# Autodesk Inventor assembly: FTC Drivetrain V1
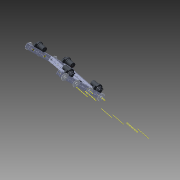
[picture p0: Inventor's stored thumbnail of the model, 180x180]
Saved by Autodesk Inventor 2015 (Build 190159000, 159)
## iProperties
Created: 2014-08-16
Part Number: FTC Drivetrain V1
Document SubType Name: Assembly
Designer: Vinay
Author: Vinay
## Documents named in this file (17)
- C:\Working Folder\FTC Drivetrain V1.iam
- C:\Working Folder\CAD Models\Imported Components\Pitsco Education-739069\Pitsco Education-739069.ipt
- C:\Working Folder\CAD Models\FTC_Tetrix_KOP_Block_Party\Tetrix_Kit_FTC\Imported Components\tetrix_739089_2012\tetrix_739089_2012.ipt
- C:\Working Folder\CAD Models\FTC_Tetrix_KOP_Block_Party\Tetrix_Kit_FTC\Imported Components\tetrix_739083_motor_2012\tetrix_739083_motor_2012.ipt
- C:\Working Folder\CAD Models\Imported Components\Pitsco Education-739091\Pitsco Education-739091.ipt
- C:\Working Folder\CAD Models\Imported Components\Pitsco Education-739069\Pitsco Education-739069_MIR.ipt
- C:\Working Folder\CAD Models\FTC_Tetrix_KOP_Block_Party\Tetrix_Kit_FTC\Imported Components\tetrix_739089_2012\tetrix_739089_2012_MIR.ipt
- C:\Working Folder\CAD Models\FTC_Tetrix_KOP_Block_Party\Tetrix_Kit_FTC\Imported Components\tetrix_739083_motor_2012\tetrix_739083_motor_2012_MIR.ipt
- C:\Working Folder\CAD Models\Imported Components\Pitsco Education-739091\Pitsco Education-739091_MIR.ipt
- C:\Working Folder\CAD Models\FTC_Tetrix_KOP_Block_Party\Tetrix_Kit_FTC\Imported Components\tetrix_739062_2012\tetrix_739062_2012.ipt
- C:\Working Folder\CAD Models\Imported Components\Pitsco Education-739068\Pitsco Education-739068.ipt
- C:\Working Folder\CAD Models\FTC_Tetrix_KOP_Block_Party\Tetrix_Kit_FTC\Imported Components\tetrix_739088_2013\tetrix_739088_2013.ipt
- C:\Working Folder\CAD Models\FTC_Tetrix_KOP_Block_Party\Tetrix_Kit_FTC\Imported Components\tetrix_739079_2012\tetrix_739079_2012.iam
- C:\Working Folder\CAD Models\FTC_Tetrix_KOP_Block_Party\Tetrix_Kit_FTC\Imported Components\tetrix_739172_2012\tetrix_739172_2012.iam
- C:\Working Folder\CAD Models\Imported Components\Pitsco Education-739169\Pitsco Education-739169.ipt
- C:\Working Folder\CAD Models\FTC_Tetrix_KOP_Block_Party\Tetrix_Kit_FTC\Imported Components\tetrix_739165_sprk_25_16t_2013\tetrix_739165_sprk_25_16t_2013.ipt
- C:\Working Folder\CAD Models\FTC_Tetrix_KOP_Block_Party\Tetrix_Kit_FTC\Imported Components\tetrix_739092_2012\tetrix_739092_2012.iam
## Components (72 placed, 16 different names)
1. Pitsco Education-739069:1 — Mate:1, Mate:2, Mate:3, Mate:4, Mate:5, Mate:6, Mate:11, Mate:12, Mate:13, Mate:14, Mate:17, Mate:18, Mate:19, Mate:20, Mate:21, Mate:22, Mate:23, Mate:24, Mate:49, Mate:50, Mate:51, Mate:61, Mate:62, Mate:63, Mate:70, Mate:71, Mate:72, Mate:73
2. tetrix_739089_2012:1 — Mate:4, Mate:5, Mate:6, Mate:7, Flush:2
3. tetrix_739089_2012:2 — Mate:1, Mate:2, Mate:3, Mate:8, Flush:1
4. tetrix_739083_motor_2012:1 — Mate:7, Flush:2, Mate:86, Mate:87
5. tetrix_739083_motor_2012:2 — Mate:8, Flush:1, Mate:88, Mate:89
6. Pitsco Education-739091:1 — Mate:11, Mate:12, Mate:134, Mate:135
7. Pitsco Education-739091:3 — Mate:13, Mate:14, Mate:85, Mate:94
8. Pitsco Education-739091:4 — Mate:72, Mate:73, Mate:82, Mate:100
9. Pitsco Education-739091:5 — Mate:23, Mate:24, Mate:146, Mate:147
10. Pitsco Education-739091:6 — Mate:70, Mate:71, Mate:84, Mate:96
11. Pitsco Education-739091:7 — Mate:21, Mate:22, Mate:142, Mate:143
12. Pitsco Education-739091:10 — Mate:19, Mate:20, Mate:136, Mate:137
13. Pitsco Education-739091:11 — Mate:17, Mate:18, Mate:83, Mate:98
14. Pitsco Education-739069_MIR:1 — Mate:25, Mate:26, Mate:27, Mate:28, Mate:29, Mate:30, Mate:33, Mate:34, Mate:35, Mate:36, Mate:39, Mate:40, Mate:43, Mate:44, Mate:45, Mate:46, Mate:47, Mate:48, Mate:58, Mate:59, Mate:60, Mate:74, Mate:75, Mate:76, Mate:77
15. tetrix_739089_2012_MIR:1 — Mate:25, Mate:26, Mate:27, Flush:3, Mate:31
16. tetrix_739089_2012_MIR:2 — Mate:28, Mate:29, Mate:30, Flush:4, Mate:32
17. tetrix_739083_motor_2012_MIR:1 — Flush:3, Mate:31, Mate:90, Mate:91
18. tetrix_739083_motor_2012_MIR:2 — Flush:4, Mate:32, Mate:92, Mate:93
19. Pitsco Education-739091_MIR:1 — Mate:33, Mate:34, Mate:140, Mate:141
20. Pitsco Education-739091_MIR:2 — Mate:35, Mate:36, Mate:81, Mate:108
21. Pitsco Education-739091_MIR:3 — Mate:76, Mate:77, Mate:78, Mate:106
22. Pitsco Education-739091_MIR:4 — Mate:39, Mate:40, Mate:148, Mate:149
23. Pitsco Education-739091_MIR:5 — Mate:74, Mate:75, Mate:80, Mate:102
24. Pitsco Education-739091_MIR:6 — Mate:43, Mate:44, Mate:144, Mate:145
25. Pitsco Education-739091_MIR:7 — Mate:45, Mate:46, Mate:138, Mate:139
26. Pitsco Education-739091_MIR:8 — Mate:47, Mate:48, Mate:79, Mate:104
27. tetrix_739062_2012:2 — Mate:49, Mate:50, Mate:51, Mate:52, Mate:53, Mate:54
28. Pitsco Education-739068:1 — Mate:52, Mate:53, Mate:54, Mate:55, Mate:56, Mate:57
29. tetrix_739062_2012:5 — Mate:55, Mate:56, Mate:57, Mate:58, Mate:59, Mate:60
30. tetrix_739062_2012:6 — Mate:61, Mate:62, Mate:63, Mate:64, Mate:65, Mate:66
31. tetrix_739062_2012:7 — Mate:67, Mate:68, Mate:69
32. Pitsco Education-739068:2 — Mate:64, Mate:65, Mate:66, Mate:67, Mate:68, Mate:69
33. tetrix_739088_2013:1 — Mate:81, Mate:109, Cylindrical:1
34. tetrix_739088_2013:2 — Mate:80, Mate:103, Mate:150
35. tetrix_739088_2013:3 — Mate:79, Mate:105
36. tetrix_739088_2013:4 — Mate:78, Mate:107
37. tetrix_739088_2013:5 — Mate:85, Mate:95
38. tetrix_739088_2013:6 — Mate:84, Mate:97
39. tetrix_739088_2013:7 — Mate:83, Mate:99
40. tetrix_739088_2013:8 — Mate:82, Mate:101
41. tetrix_739079_2012:1 [sub-assembly] — Mate:88, Mate:89, Mate:112, Mate:113
42. tetrix_739079_2012:2 [sub-assembly] — Mate:86, Mate:87, Mate:116, Mate:117
43. tetrix_739079_2012:3 [sub-assembly] — Mate:92, Mate:93, Mate:122, Mate:123
44. tetrix_739079_2012:4 [sub-assembly] — Mate:90, Mate:91, Mate:132, Mate:133
45. tetrix_739172_2012:1 [sub-assembly] — Mate:94, Mate:95, Mate:110, Mate:111
46. tetrix_739172_2012:2 [sub-assembly] — Mate:100, Mate:101, Mate:120, Mate:121
47. tetrix_739172_2012:3 [sub-assembly] — Mate:98, Mate:99, Mate:118, Mate:119
48. tetrix_739172_2012:4 [sub-assembly] — Mate:96, Mate:97, Mate:114, Mate:115
49. tetrix_739172_2012:5 [sub-assembly] — Mate:102, Mate:103, Mate:128, Mate:129
50. tetrix_739172_2012:6 [sub-assembly] — Mate:104, Mate:105, Mate:126, Mate:127
51. tetrix_739172_2012:7 [sub-assembly] — Mate:106, Mate:107, Mate:124, Mate:125
52. tetrix_739172_2012:8 [sub-assembly] — Mate:108, Mate:109, Mate:130, Mate:131
53. Pitsco Education-739169:1 — Mate:110, Mate:111
54. Pitsco Education-739169:2 — Mate:114, Mate:115
55. Pitsco Education-739169:3 — Mate:118, Mate:119
56. Pitsco Education-739169:4 — Mate:120, Mate:121
57. tetrix_739165_sprk_25_16t_2013:1 — Mate:122, Mate:123
58. tetrix_739165_sprk_25_16t_2013:2 — Mate:112, Mate:113
59. tetrix_739165_sprk_25_16t_2013:3 — Mate:116, Mate:117
60. Pitsco Education-739169:5 — Mate:124, Mate:125
61. Pitsco Education-739169:6 — Mate:126, Mate:127
62. Pitsco Education-739169:7 — Mate:130, Mate:131, Cylindrical:1
63. Pitsco Education-739169:8 — Mate:128, Mate:129
64. tetrix_739165_sprk_25_16t_2013:4 — Mate:132, Mate:133
65. tetrix_739092_2012:1 [sub-assembly] — Mate:138, Mate:139
66. tetrix_739092_2012:2 [sub-assembly] — Mate:142, Mate:143
67. tetrix_739092_2012:3 [sub-assembly] — Mate:140, Mate:141
68. tetrix_739092_2012:4 [sub-assembly] — Mate:146, Mate:147
69. tetrix_739092_2012:5 [sub-assembly] — Mate:136, Mate:137
70. tetrix_739092_2012:6 [sub-assembly] — Mate:144, Mate:145, Mate:150
71. tetrix_739092_2012:7 [sub-assembly] — Mate:148, Mate:149
72. tetrix_739092_2012:8 [sub-assembly] — Mate:134, Mate:135
## Relationships (147: Mate 142, Flush 4, CylindricalJoint 1)
- Mate:1: Pitsco Education-739069:1 ↔ tetrix_739089_2012:2
- Mate:2: Pitsco Education-739069:1 ↔ tetrix_739089_2012:2
- Mate:3: Pitsco Education-739069:1 ↔ tetrix_739089_2012:2
- Mate:4: Pitsco Education-739069:1 ↔ tetrix_739089_2012:1
- Mate:5: Pitsco Education-739069:1 ↔ tetrix_739089_2012:1
- Mate:6: Pitsco Education-739069:1 ↔ tetrix_739089_2012:1
- Mate:7: tetrix_739089_2012:1 ↔ tetrix_739083_motor_2012:1
- Mate:8: tetrix_739089_2012:2 ↔ tetrix_739083_motor_2012:2
- Flush:1: tetrix_739089_2012:2 ↔ tetrix_739083_motor_2012:2
- Flush:2: tetrix_739089_2012:1 ↔ tetrix_739083_motor_2012:1
- Mate:11: Pitsco Education-739069:1 ↔ Pitsco Education-739091:1
- Mate:12: Pitsco Education-739069:1 ↔ Pitsco Education-739091:1
- Mate:13: Pitsco Education-739069:1 ↔ Pitsco Education-739091:3
- Mate:14: Pitsco Education-739069:1 ↔ Pitsco Education-739091:3
- Mate:17: Pitsco Education-739069:1 ↔ Pitsco Education-739091:11
- Mate:18: Pitsco Education-739069:1 ↔ Pitsco Education-739091:11
- Mate:19: Pitsco Education-739069:1 ↔ Pitsco Education-739091:10
- Mate:20: Pitsco Education-739069:1 ↔ Pitsco Education-739091:10
- Mate:21: Pitsco Education-739069:1 ↔ Pitsco Education-739091:7
- Mate:22: Pitsco Education-739069:1 ↔ Pitsco Education-739091:7
- Mate:23: Pitsco Education-739069:1 ↔ Pitsco Education-739091:5
- Mate:24: Pitsco Education-739069:1 ↔ Pitsco Education-739091:5
- Mate:25: Pitsco Education-739069_MIR:1 ↔ tetrix_739089_2012_MIR:1
- Mate:26: Pitsco Education-739069_MIR:1 ↔ tetrix_739089_2012_MIR:1
- Mate:27: Pitsco Education-739069_MIR:1 ↔ tetrix_739089_2012_MIR:1
- Mate:28: Pitsco Education-739069_MIR:1 ↔ tetrix_739089_2012_MIR:2
- Mate:29: Pitsco Education-739069_MIR:1 ↔ tetrix_739089_2012_MIR:2
- Mate:30: Pitsco Education-739069_MIR:1 ↔ tetrix_739089_2012_MIR:2
- Flush:3: tetrix_739089_2012_MIR:1 ↔ tetrix_739083_motor_2012_MIR:1
- Mate:31: tetrix_739089_2012_MIR:1 ↔ tetrix_739083_motor_2012_MIR:1
- Flush:4: tetrix_739089_2012_MIR:2 ↔ tetrix_739083_motor_2012_MIR:2
- Mate:32: tetrix_739089_2012_MIR:2 ↔ tetrix_739083_motor_2012_MIR:2
- Mate:33: Pitsco Education-739069_MIR:1 ↔ Pitsco Education-739091_MIR:1
- Mate:34: Pitsco Education-739069_MIR:1 ↔ Pitsco Education-739091_MIR:1
- Mate:35: Pitsco Education-739069_MIR:1 ↔ Pitsco Education-739091_MIR:2
- Mate:36: Pitsco Education-739069_MIR:1 ↔ Pitsco Education-739091_MIR:2
- Mate:39: Pitsco Education-739069_MIR:1 ↔ Pitsco Education-739091_MIR:4
- Mate:40: Pitsco Education-739069_MIR:1 ↔ Pitsco Education-739091_MIR:4
- Mate:43: Pitsco Education-739069_MIR:1 ↔ Pitsco Education-739091_MIR:6
- Mate:44: Pitsco Education-739069_MIR:1 ↔ Pitsco Education-739091_MIR:6
- Mate:45: Pitsco Education-739069_MIR:1 ↔ Pitsco Education-739091_MIR:7
- Mate:46: Pitsco Education-739069_MIR:1 ↔ Pitsco Education-739091_MIR:7
- Mate:47: Pitsco Education-739069_MIR:1 ↔ Pitsco Education-739091_MIR:8
- Mate:48: Pitsco Education-739069_MIR:1 ↔ Pitsco Education-739091_MIR:8
- Mate:49: Pitsco Education-739069:1 ↔ tetrix_739062_2012:2
- Mate:50: Pitsco Education-739069:1 ↔ tetrix_739062_2012:2
- Mate:51: Pitsco Education-739069:1 ↔ tetrix_739062_2012:2
- Mate:52: tetrix_739062_2012:2 ↔ Pitsco Education-739068:1
- Mate:53: tetrix_739062_2012:2 ↔ Pitsco Education-739068:1
- Mate:54: tetrix_739062_2012:2 ↔ Pitsco Education-739068:1
- Mate:55: Pitsco Education-739068:1 ↔ tetrix_739062_2012:5
- Mate:56: Pitsco Education-739068:1 ↔ tetrix_739062_2012:5
- Mate:57: Pitsco Education-739068:1 ↔ tetrix_739062_2012:5
- Mate:58: Pitsco Education-739069_MIR:1 ↔ tetrix_739062_2012:5
- Mate:59: Pitsco Education-739069_MIR:1 ↔ tetrix_739062_2012:5
- Mate:60: Pitsco Education-739069_MIR:1 ↔ tetrix_739062_2012:5
- Mate:61: Pitsco Education-739069:1 ↔ tetrix_739062_2012:6
- Mate:62: Pitsco Education-739069:1 ↔ tetrix_739062_2012:6
- Mate:63: Pitsco Education-739069:1 ↔ tetrix_739062_2012:6
- Mate:64: tetrix_739062_2012:6 ↔ Pitsco Education-739068:2
- Mate:65: tetrix_739062_2012:6 ↔ Pitsco Education-739068:2
- Mate:66: tetrix_739062_2012:6 ↔ Pitsco Education-739068:2
- Mate:67: tetrix_739062_2012:7 ↔ Pitsco Education-739068:2
- Mate:68: tetrix_739062_2012:7 ↔ Pitsco Education-739068:2
- Mate:69: tetrix_739062_2012:7 ↔ Pitsco Education-739068:2
- Mate:70: Pitsco Education-739069:1 ↔ Pitsco Education-739091:6
- Mate:71: Pitsco Education-739069:1 ↔ Pitsco Education-739091:6
- Mate:72: Pitsco Education-739069:1 ↔ Pitsco Education-739091:4
- Mate:73: Pitsco Education-739069:1 ↔ Pitsco Education-739091:4
- Mate:74: Pitsco Education-739069_MIR:1 ↔ Pitsco Education-739091_MIR:5
- Mate:75: Pitsco Education-739069_MIR:1 ↔ Pitsco Education-739091_MIR:5
- Mate:76: Pitsco Education-739069_MIR:1 ↔ Pitsco Education-739091_MIR:3
- Mate:77: Pitsco Education-739069_MIR:1 ↔ Pitsco Education-739091_MIR:3
- Mate:78: Pitsco Education-739091_MIR:3 ↔ tetrix_739088_2013:4
- Mate:79: Pitsco Education-739091_MIR:8 ↔ tetrix_739088_2013:3
- Mate:80: Pitsco Education-739091_MIR:5 ↔ tetrix_739088_2013:2
- Mate:81: Pitsco Education-739091_MIR:2 ↔ tetrix_739088_2013:1
- Mate:82: Pitsco Education-739091:4 ↔ tetrix_739088_2013:8
- Mate:83: Pitsco Education-739091:11 ↔ tetrix_739088_2013:7
- Mate:84: Pitsco Education-739091:6 ↔ tetrix_739088_2013:6
- Mate:85: Pitsco Education-739091:3 ↔ tetrix_739088_2013:5
- Mate:86: tetrix_739083_motor_2012:1 ↔ tetrix_739079_2012:2
- Mate:87: tetrix_739083_motor_2012:1 ↔ tetrix_739079_2012:2
- Mate:88: tetrix_739083_motor_2012:2 ↔ tetrix_739079_2012:1
- Mate:89: tetrix_739083_motor_2012:2 ↔ tetrix_739079_2012:1
- Mate:90: tetrix_739083_motor_2012_MIR:1 ↔ tetrix_739079_2012:4
- Mate:91: tetrix_739083_motor_2012_MIR:1 ↔ tetrix_739079_2012:4
- Mate:92: tetrix_739083_motor_2012_MIR:2 ↔ tetrix_739079_2012:3
- Mate:93: tetrix_739083_motor_2012_MIR:2 ↔ tetrix_739079_2012:3
- Mate:94: Pitsco Education-739091:3 ↔ tetrix_739172_2012:1
- Mate:95: tetrix_739088_2013:5 ↔ tetrix_739172_2012:1
- Mate:96: Pitsco Education-739091:6 ↔ tetrix_739172_2012:4
- Mate:97: tetrix_739088_2013:6 ↔ tetrix_739172_2012:4
- Mate:98: Pitsco Education-739091:11 ↔ tetrix_739172_2012:3
- Mate:99: tetrix_739088_2013:7 ↔ tetrix_739172_2012:3
- Mate:100: Pitsco Education-739091:4 ↔ tetrix_739172_2012:2
- Mate:101: tetrix_739088_2013:8 ↔ tetrix_739172_2012:2
- Mate:102: Pitsco Education-739091_MIR:5 ↔ tetrix_739172_2012:5
- Mate:103: tetrix_739088_2013:2 ↔ tetrix_739172_2012:5
- Mate:104: Pitsco Education-739091_MIR:8 ↔ tetrix_739172_2012:6
- Mate:105: tetrix_739088_2013:3 ↔ tetrix_739172_2012:6
- Mate:106: Pitsco Education-739091_MIR:3 ↔ tetrix_739172_2012:7
- Mate:107: tetrix_739088_2013:4 ↔ tetrix_739172_2012:7
- Mate:108: Pitsco Education-739091_MIR:2 ↔ tetrix_739172_2012:8
- Mate:109: tetrix_739088_2013:1 ↔ tetrix_739172_2012:8
- Mate:110: tetrix_739172_2012:1 ↔ Pitsco Education-739169:1
- Mate:111: tetrix_739172_2012:1 ↔ Pitsco Education-739169:1
- Mate:112: tetrix_739079_2012:1 ↔ tetrix_739165_sprk_25_16t_2013:2
- Mate:113: tetrix_739079_2012:1 ↔ tetrix_739165_sprk_25_16t_2013:2
- Mate:114: tetrix_739172_2012:4 ↔ Pitsco Education-739169:2
- Mate:115: tetrix_739172_2012:4 ↔ Pitsco Education-739169:2
- Mate:116: tetrix_739079_2012:2 ↔ tetrix_739165_sprk_25_16t_2013:3
- Mate:117: tetrix_739079_2012:2 ↔ tetrix_739165_sprk_25_16t_2013:3
- Mate:118: tetrix_739172_2012:3 ↔ Pitsco Education-739169:3
- Mate:119: tetrix_739172_2012:3 ↔ Pitsco Education-739169:3
- Mate:120: tetrix_739172_2012:2 ↔ Pitsco Education-739169:4
- Mate:121: tetrix_739172_2012:2 ↔ Pitsco Education-739169:4
- Mate:122: tetrix_739079_2012:3 ↔ tetrix_739165_sprk_25_16t_2013:1
- Mate:123: tetrix_739079_2012:3 ↔ tetrix_739165_sprk_25_16t_2013:1
- Mate:124: tetrix_739172_2012:7 ↔ Pitsco Education-739169:5
- Mate:125: tetrix_739172_2012:7 ↔ Pitsco Education-739169:5
- Mate:126: tetrix_739172_2012:6 ↔ Pitsco Education-739169:6
- Mate:127: tetrix_739172_2012:6 ↔ Pitsco Education-739169:6
- Mate:128: tetrix_739172_2012:5 ↔ Pitsco Education-739169:8
- Mate:129: tetrix_739172_2012:5 ↔ Pitsco Education-739169:8
- Mate:130: tetrix_739172_2012:8 ↔ Pitsco Education-739169:7
- Mate:131: tetrix_739172_2012:8 ↔ Pitsco Education-739169:7
- Mate:132: tetrix_739079_2012:4 ↔ tetrix_739165_sprk_25_16t_2013:4
- Mate:133: tetrix_739079_2012:4 ↔ tetrix_739165_sprk_25_16t_2013:4
- Mate:134: Pitsco Education-739091:1 ↔ tetrix_739092_2012:8
- Mate:135: Pitsco Education-739091:1 ↔ tetrix_739092_2012:8
- Mate:136: Pitsco Education-739091:10 ↔ tetrix_739092_2012:5
- Mate:137: Pitsco Education-739091:10 ↔ tetrix_739092_2012:5
- Mate:138: Pitsco Education-739091_MIR:7 ↔ tetrix_739092_2012:1
- Mate:139: Pitsco Education-739091_MIR:7 ↔ tetrix_739092_2012:1
- Mate:140: Pitsco Education-739091_MIR:1 ↔ tetrix_739092_2012:3
- Mate:141: Pitsco Education-739091_MIR:1 ↔ tetrix_739092_2012:3
- Mate:142: Pitsco Education-739091:7 ↔ tetrix_739092_2012:2
- Mate:143: Pitsco Education-739091:7 ↔ tetrix_739092_2012:2
- Mate:144: Pitsco Education-739091_MIR:6 ↔ tetrix_739092_2012:6
- Mate:145: Pitsco Education-739091_MIR:6 ↔ tetrix_739092_2012:6
- Mate:146: Pitsco Education-739091:5 ↔ tetrix_739092_2012:4
- Mate:147: Pitsco Education-739091:5 ↔ tetrix_739092_2012:4
- Mate:148: Pitsco Education-739091_MIR:4 ↔ tetrix_739092_2012:7
- Mate:149: Pitsco Education-739091_MIR:4 ↔ tetrix_739092_2012:7
- Cylindrical:1: tetrix_739088_2013:1 ↔ Pitsco Education-739169:7
- Mate:150: tetrix_739088_2013:2 ↔ tetrix_739092_2012:6
